# Autodesk Inventor assembly: mg996r_left_top_rot_frame
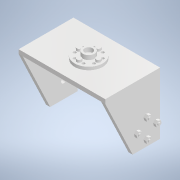
[picture p0: Inventor's stored thumbnail of the model, 180x180]
Saved by Autodesk Inventor 2021.4 (Build 254397000, 397)
## iProperties
Created: 2022-07-25
Part Number: mg996r_left_top_rot_frame
Document SubType Name: Assembly
Designer: isamu
Author: isamu
## Documents named in this file (6)
- D:\personal_projects\robot\inventor\2021_matlab_compat\mg996r_left_top_rot_frame.iam
- D:\personal_projects\robot\exports\handle\servo handle 4.ipt
- D:\personal_projects\robot\exports\frames\servo frame mg996 centered.ipt
- D:\personal_projects\robot\exports\screws\m4 nuts.ipt
- D:\personal_projects\robot\exports\screws\m2x8.ipt
- D:\personal_projects\robot\exports\screws\m2 nuts.ipt
## Components (20 placed, 5 different names)
1. servo handle 4:1 — Mate:1, Mate:2, Mate:3, Insert:2, Insert:3, Insert:4, Insert:5
2. servo frame mg996 centered:1 — Mate:1, Mate:2, Mate:3, Insert:1, Insert:6, Insert:7, Insert:8, Insert:9, Mate:4, Mate:5, Mate:6, Insert:14, Insert:15, Insert:16, Insert:17
3. m4 nuts:1 — Insert:1
4. m2x8:1 — Insert:5
5. m2x8:2 — Insert:3
6. m2x8:3 — Insert:2
7. m2x8:4 — Insert:4
8. m2 nuts:1 — Insert:6
9. m2 nuts:2 — Insert:7
10. m2 nuts:3 — Insert:8
11. m2 nuts:4 — Insert:9
12. m2x8:5 — Insert:13
13. m2x8:6 — Insert:12
14. m2x8:7 — Insert:11
15. m2x8:8 — Insert:10
16. m2 nuts:5 — Insert:16
17. m2 nuts:6 — Insert:15
18. m2 nuts:7 — Insert:17
19. m2 nuts:8 — Insert:14
20. servo handle 4:2 — Mate:4, Mate:5, Mate:6, Insert:10, Insert:11, Insert:12, Insert:13
## Relationships (23: Insert 17, Mate 6)
- Mate:1: servo handle 4:1 ↔ servo frame mg996 centered:1
- Mate:2: servo handle 4:1 ↔ servo frame mg996 centered:1
- Mate:3: servo handle 4:1 ↔ servo frame mg996 centered:1
- Insert:1: servo frame mg996 centered:1 ↔ m4 nuts:1
- Insert:2: servo handle 4:1 ↔ m2x8:3
- Insert:3: servo handle 4:1 ↔ m2x8:2
- Insert:4: servo handle 4:1 ↔ m2x8:4
- Insert:5: servo handle 4:1 ↔ m2x8:1
- Insert:6: servo frame mg996 centered:1 ↔ m2 nuts:1
- Insert:7: servo frame mg996 centered:1 ↔ m2 nuts:2
- Insert:8: servo frame mg996 centered:1 ↔ m2 nuts:3
- Insert:9: servo frame mg996 centered:1 ↔ m2 nuts:4
- Mate:4: servo frame mg996 centered:1 ↔ servo handle 4:2
- Mate:5: servo frame mg996 centered:1 ↔ servo handle 4:2
- Mate:6: servo frame mg996 centered:1 ↔ servo handle 4:2
- Insert:10: m2x8:8 ↔ servo handle 4:2
- Insert:11: m2x8:7 ↔ servo handle 4:2
- Insert:12: m2x8:6 ↔ servo handle 4:2
- Insert:13: m2x8:5 ↔ servo handle 4:2
- Insert:14: servo frame mg996 centered:1 ↔ m2 nuts:8
- Insert:15: servo frame mg996 centered:1 ↔ m2 nuts:6
- Insert:16: servo frame mg996 centered:1 ↔ m2 nuts:5
- Insert:17: servo frame mg996 centered:1 ↔ m2 nuts:7
